# Autodesk Inventor assembly: Wózek_inwalidzki
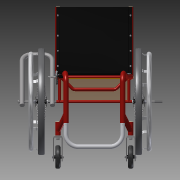
[picture p0: Inventor's stored thumbnail of the model, 180x180]
Saved by Autodesk Inventor 2015 (Build 190159000, 159)
## iProperties
Created: 2016-01-12
Part Number: Wózek_inwalidzki
Document SubType Name: Assembly
Designer: graaapsik
Author: graaapsik
## Documents named in this file (14)
- C:\Users\EriveltonDell\Documents\Centro Universitário da FEI\Wheelchair\CADEIRA DE RODAS - DESENHO\Model\Wózek_inwalidzki.iam
- C:\Users\EriveltonDell\Documents\Centro Universitário da FEI\Wheelchair\CADEIRA DE RODAS - DESENHO\Model\Hamulec.iam
- C:\Users\EriveltonDell\Documents\Centro Universitário da FEI\Wheelchair\CADEIRA DE RODAS - DESENHO\Model\Koło_przednie.iam
- C:\Users\EriveltonDell\Documents\Centro Universitário da FEI\Wheelchair\CADEIRA DE RODAS - DESENHO\Model\Koło_tylne.iam
- C:\Users\EriveltonDell\Documents\Centro Universitário da FEI\Wheelchair\CADEIRA DE RODAS - DESENHO\Model\Rama_wozka.iam
- C:\Users\EriveltonDell\Documents\Centro Universitário da FEI\Wheelchair\CADEIRA DE RODAS - DESENHO\Model\Tapicerka_oparcia.iam
- C:\Users\EriveltonDell\Documents\Centro Universitário da FEI\Wheelchair\CADEIRA DE RODAS - DESENHO\Model\Tapicerka_siedziska.iam
- C:\Users\EriveltonDell\Documents\Centro Universitário da FEI\Wheelchair\CADEIRA DE RODAS - DESENHO\Model\Ciąg.iam
- C:\Users\EriveltonDell\Documents\Centro Universitário da FEI\Wheelchair\CADEIRA DE RODAS - DESENHO\Model\Widelec.iam
- C:\Users\EriveltonDell\Documents\Centro Universitário da FEI\Wheelchair\CADEIRA DE RODAS - DESENHO\Model\Zaślepka_do_widelca.ipt
- C:\Users\EriveltonDell\Documents\Centro Universitário da FEI\Wheelchair\CADEIRA DE RODAS - DESENHO\Model\Podnóżek.iam
- C:\Users\EriveltonDell\Documents\Centro Universitário da FEI\Wheelchair\CADEIRA DE RODAS - DESENHO\Model\Zaślepka_do_rur_fi32.ipt
- C:\Users\EriveltonDell\Documents\Centro Universitário da FEI\Wheelchair\CADEIRA DE RODAS - DESENHO\Model\GARFO.ipt
- C:\Users\EriveltonDell\Documents\Centro Universitário da FEI\Wheelchair\CADEIRA DE RODAS - DESENHO\Model\ISO 4032 - M10ISO.ipt
## Components (21 placed, 13 different names)
1. Rama_wozka:1 [sub-assembly] — Zestawiający:1, Zestawiający:2, Zestawiający:7, Zestawiający:8, Zestawiający:9, Zestawiający:10, Zestawiający:11, Zestawiający:12, Równoległy:1, Zestawiający:15, Symetria:1, Równoległy:2, Zestawiający:20, Zestawiający:22, Wstaw:1, Zestawiający:27, Zestawiający:29, Wstaw:2, Zestawiający:36, Zestawiający:37, Równoległy:3, Zestawiający:38, Zestawiający:39, Zestawiający:40, Zestawiający:41, Zestawiający:42, Zestawiający:43, Zestawiający:44, Zestawiający:45
2. Koło_tylne:1 [sub-assembly] — Zestawiający:1, Wstaw:1, Zestawiający:24, Zestawiający:25, Styczny:1, Kąt:1, Mate:46, Tangent:2, Insert:4
3. Koło_tylne:2 [sub-assembly] — Zestawiający:2, Wstaw:2, Zestawiający:30, Zestawiający:31, Kąt:2
4. Ciąg:1 [sub-assembly] — Zestawiający:30, Zestawiający:31
5. Ciąg:2 [sub-assembly] — Zestawiający:24, Zestawiający:25
6. Widelec:1 [sub-assembly] — Zestawiający:9, Zestawiający:11, Wstaw:3
7. Widelec:2 [sub-assembly] — Zestawiający:10, Zestawiający:12, Zestawiający:13, Zestawiający:14, Symetria:1
8. Koło_przednie:1 [sub-assembly] — Wstaw:3, Kąt:1
9. Koło_przednie:2 [sub-assembly] — Zestawiający:13, Zestawiający:14, Kąt:2
10. Hamulec:1 [sub-assembly] — Zestawiający:38, Zestawiający:39, Styczny:1
11. Tapicerka_oparcia:1 [sub-assembly] — Równoległy:1, Zestawiający:16
12. Tapicerka_siedziska:1 [sub-assembly] — Zestawiający:15, Zestawiający:16
13. Zaślepka_do_widelca:1 — Zestawiający:8, Zestawiający:45
14. Zaślepka_do_widelca:2 — Zestawiający:7, Zestawiający:44
15. Podnóżek:1 [sub-assembly] — Zestawiający:36, Zestawiający:37, Równoległy:3
16. Zaślepka_do_rur_fi32:1 — Zestawiający:22, Zestawiający:42
17. Zaślepka_do_rur_fi32:2 — Zestawiający:27, Zestawiający:40
18. Zaślepka_do_rur_fi32:3 — Zestawiający:20, Zestawiający:43
19. Zaślepka_do_rur_fi32:5 — Zestawiający:29, Zestawiający:41
20. GARFO:1 — Mate:46, Tangent:2
21. ISO 4032 M10:1 — Insert:4
## Relationships (43: Mate 31, Insert 4, Flush 3, Tangent 2, Angle 2, Symmetry 1)
- Zestawiający:1 [Mate]: Rama_wozka:1 ↔ Koło_tylne:1
- Zestawiający:2 [Mate]: Rama_wozka:1 ↔ Koło_tylne:2
- Zestawiający:7 [Mate]: Rama_wozka:1 ↔ Zaślepka_do_widelca:2
- Zestawiający:8 [Mate]: Rama_wozka:1 ↔ Zaślepka_do_widelca:1
- Zestawiający:9 [Mate]: Rama_wozka:1 ↔ Widelec:1
- Zestawiający:10 [Mate]: Rama_wozka:1 ↔ Widelec:2
- Zestawiający:11 [Mate]: Rama_wozka:1 ↔ Widelec:1
- Zestawiający:12 [Mate]: Rama_wozka:1 ↔ Widelec:2
- Zestawiający:13 [Mate]: Widelec:2 ↔ Koło_przednie:2
- Zestawiający:14 [Mate]: Widelec:2 ↔ Koło_przednie:2
- Równoległy:1 [Flush] (-16 mm): Rama_wozka:1 ↔ Tapicerka_oparcia:1
- Zestawiający:15 [Mate] (16 mm): Rama_wozka:1 ↔ Tapicerka_siedziska:1
- Zestawiający:16 [Mate] (0.25 mm): Tapicerka_oparcia:1 ↔ Tapicerka_siedziska:1
- Symetria:1 [Symmetry]: Rama_wozka:1 ↔ Widelec:2
- Równoległy:2 [Flush]: Rama_wozka:1
- Zestawiający:20 [Mate]: Rama_wozka:1 ↔ Zaślepka_do_rur_fi32:3
- Zestawiający:22 [Mate]: Rama_wozka:1 ↔ Zaślepka_do_rur_fi32:1
- Wstaw:1 [Insert] (50 mm): Rama_wozka:1 ↔ Koło_tylne:1
- Zestawiający:24 [Mate]: Koło_tylne:1 ↔ Ciąg:2
- Zestawiający:25 [Mate]: Koło_tylne:1 ↔ Ciąg:2
- Zestawiający:27 [Mate]: Rama_wozka:1 ↔ Zaślepka_do_rur_fi32:2
- Zestawiający:29 [Mate]: Rama_wozka:1 ↔ Zaślepka_do_rur_fi32:5
- Wstaw:2 [Insert]: Rama_wozka:1 ↔ Koło_tylne:2
- Zestawiający:30 [Mate]: Koło_tylne:2 ↔ Ciąg:1
- Zestawiający:31 [Mate]: Koło_tylne:2 ↔ Ciąg:1
- Wstaw:3 [Insert]: Widelec:1 ↔ Koło_przednie:1
- Zestawiający:36 [Mate]: Rama_wozka:1 ↔ Podnóżek:1
- Zestawiający:37 [Mate]: Rama_wozka:1 ↔ Podnóżek:1
- Równoległy:3 [Flush] (150 mm): Rama_wozka:1 ↔ Podnóżek:1
- Zestawiający:38 [Mate]: Rama_wozka:1 ↔ Hamulec:1
- Zestawiający:39 [Mate] (40 mm): Rama_wozka:1 ↔ Hamulec:1
- Styczny:1 [Tangent]: Koło_tylne:1 ↔ Hamulec:1
- Zestawiający:40 [Mate]: Rama_wozka:1 ↔ Zaślepka_do_rur_fi32:2
- Zestawiający:41 [Mate]: Rama_wozka:1 ↔ Zaślepka_do_rur_fi32:5
- Zestawiający:42 [Mate]: Rama_wozka:1 ↔ Zaślepka_do_rur_fi32:1
- Zestawiający:43 [Mate]: Rama_wozka:1 ↔ Zaślepka_do_rur_fi32:3
- Zestawiający:44 [Mate]: Rama_wozka:1 ↔ Zaślepka_do_widelca:2
- Zestawiający:45 [Mate]: Rama_wozka:1 ↔ Zaślepka_do_widelca:1
- Kąt:1 [Angle] (0 deg): Koło_tylne:1 ↔ Koło_przednie:1
- Kąt:2 [Angle] (0 deg): Koło_tylne:2 ↔ Koło_przednie:2
- Mate:46: Koło_tylne:1 ↔ GARFO:1
- Tangent:2: Koło_tylne:1 ↔ GARFO:1
- Insert:4: Koło_tylne:1 ↔ ISO 4032 M10:1
